# Autodesk Inventor assembly: Telescope
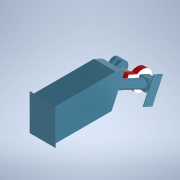
[picture p0: Inventor's stored thumbnail of the model, 180x180]
Saved by Autodesk Inventor 2022 (Build 260153000, 153)
## iProperties
Created: 2021-04-24
Part Number: Telescope
Document SubType Name: Assembly
Designer: Mick Veldhuis
Author: Mick Veldhuis
## Documents named in this file (9)
- C:\Users\Mick Veldhuis\Desktop\bsc-project\inventor\observatory\TelescopeMount.iam
- TelescopeMount.iam
- C:\Users\Mick Veldhuis\Desktop\bsc-project\inventor\observatory\Base.ipt
- C:\Users\Mick Veldhuis\Desktop\bsc-project\inventor\observatory\RaAxis.ipt
- RaAxis.ipt
- C:\Users\Mick Veldhuis\Desktop\bsc-project\inventor\observatory\AxisConnector.ipt
- C:\Users\Mick Veldhuis\Desktop\bsc-project\inventor\observatory\DecAxis.ipt
- C:\Users\Mick Veldhuis\Desktop\bsc-project\inventor\observatory\BigCounterWeight.ipt
- C:\Users\Mick Veldhuis\Desktop\bsc-project\inventor\observatory\SmallCounterWeight.ipt
## Components (7 placed, 6 different names)
1. Base:1 — RaDrive
2. RaAxis:1 — RaDrive, Mate:1, Tangent:1, Tangent:2
3. AxisConnector:1 — DecDrive, Mate:1, Tangent:1, Tangent:2, Mate:2
4. DecAxis:1 — DecDrive, Tangent:3, Insert:1, Insert:2
5. BigCounterWeight:1 — Mate:2, Tangent:3
6. SmallCounterWeight:1 — Insert:2
7. SmallCounterWeight:2 — Insert:1
## Relationships (9: Tangent 3, RevoluteJoint 2, Mate 2, Insert 2)
- RaDrive [RevoluteJoint]: Base:1 ↔ RaAxis:1
- DecDrive [RevoluteJoint] (-624 mm): AxisConnector:1 ↔ DecAxis:1
- Mate:1: RaAxis:1 ↔ AxisConnector:1
- Tangent:1: RaAxis:1 ↔ AxisConnector:1
- Tangent:2: RaAxis:1 ↔ AxisConnector:1
- Mate:2: AxisConnector:1 ↔ BigCounterWeight:1
- Tangent:3: DecAxis:1 ↔ BigCounterWeight:1
- Insert:1 (100 mm): DecAxis:1 ↔ SmallCounterWeight:2
- Insert:2 (20 mm): DecAxis:1 ↔ SmallCounterWeight:1
